# Autodesk Inventor assembly: Driver Board Mount HSI
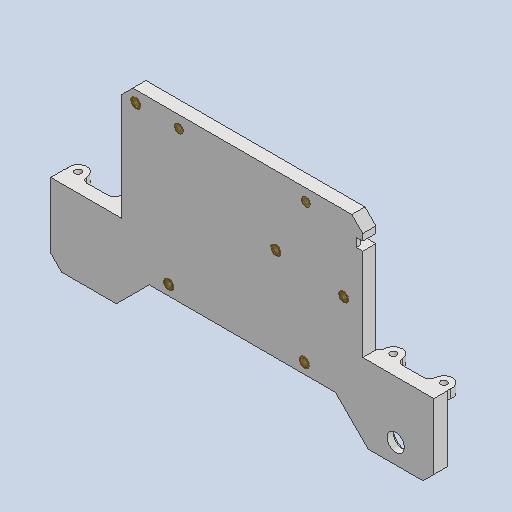
[picture p0: Inventor's stored thumbnail of the model, 512x512]
Saved by Autodesk Inventor 2022 (Build 260153000, 153)
## iProperties
Created: 2022-06-07
Part Number: Driver Board Mount HSI
Document SubType Name: Assembly
Designer: Nick
Author: Nick
## Documents named in this file (3)
- Y:\Projects\Mini_Sand_Table\Driver Board Mount HSI.iam
- Y:\Projects\Mini_Sand_Table\Motor Side Foot.ipt
- Y:\Projects\Mini_Sand_Table\M3 Heat Set Inserts.ipt
## Components (8 placed, 2 different names)
1. Motor Side Foot:1 — Insert:1, Insert:2, Insert:3, Insert:4, Insert:5, Insert:6, Insert:7
2. M3 Heat Set Inserts:1 — Insert:1
3. M3 Heat Set Inserts:2 — Insert:3
4. M3 Heat Set Inserts:3 — Insert:2
5. M3 Heat Set Inserts:4 — Insert:4
6. M3 Heat Set Inserts:5 — Insert:5
7. M3 Heat Set Inserts:6 — Insert:6
8. M3 Heat Set Inserts:7 — Insert:7
## Relationships (7: Insert 7)
- Insert:1: Motor Side Foot:1 ↔ M3 Heat Set Inserts:1
- Insert:2: Motor Side Foot:1 ↔ M3 Heat Set Inserts:3
- Insert:3: Motor Side Foot:1 ↔ M3 Heat Set Inserts:2
- Insert:4: Motor Side Foot:1 ↔ M3 Heat Set Inserts:4
- Insert:5: Motor Side Foot:1 ↔ M3 Heat Set Inserts:5
- Insert:6: Motor Side Foot:1 ↔ M3 Heat Set Inserts:6
- Insert:7: Motor Side Foot:1 ↔ M3 Heat Set Inserts:7
